# Autodesk Inventor assembly: MBD_Lupframe
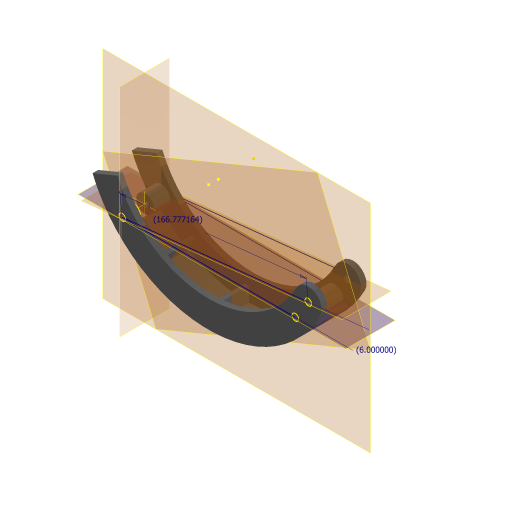
[picture p0: Inventor's stored thumbnail of the model, 512x512]
Saved by Autodesk Inventor 2023 (Build 270158000, 158)
## iProperties
Created: 2022-06-22
Part Number: MBD_Lupframe
Document SubType Name: Assembly
Designer: BioRoLaT470S
Author: BioRoLaT470S
## Documents named in this file (2)
- C:\Users\guanlunlu\Desktop\MBD_CORGI\CAD\MBD_Lupframe.iam
- C:\Users\guanlunlu\Desktop\MBD_CORGI\R100_properties\組合檔_v4\upframe_R100_v2.ipt
## Components (1 placed, 1 different names)
1. upframe_R100_v2:1 — Mate:1, Mate:2, Flush:1
## Relationships (3: Mate 2, Flush 1)
- Mate:1: upframe_R100_v2:1
- Mate:2: upframe_R100_v2:1
- Flush:1: upframe_R100_v2:1
